# Autodesk Inventor assembly: wheel single_MIR
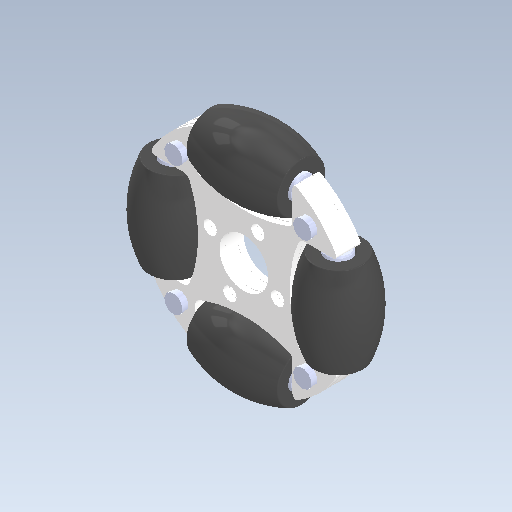
[picture p0: Inventor's stored thumbnail of the model, 512x512]
Saved by Autodesk Inventor 2020 (Build 240168000, 168)
## iProperties
Created: 2019-10-31
Part Number: wheel single_MIR
Document SubType Name: Assembly
Designer: jackm
Author: ball
Revision Number: ÈÎºÎ
## Documents named in this file (7)
- D:\FTC8863\2019 Robot\Odoemetry module\wheel single_MIR.iam
- D:\FTC8863\2019 Robot\Odoemetry module\1.5´ç90¶ÈÂÖ¹Ì¶¨°å_MIR1.ipt
- D:\FTC8863\2019 Robot\Odoemetry module\1.5´ç90¶ÈÂÖ¹Ì¶¨±ßÆ¬_MIR1.ipt
- D:\FTC8863\2019 Robot\Odoemetry module\1.5´ç90¶ÈÂÖÐ¡ÂÖÖá_MIR1.ipt
- D:\FTC8863\2019 Robot\Odoemetry module\1.5´ç90¶È»¡ÐÎÂÖ_MIR1.ipt
- D:\FTC8863\2019 Robot\Odoemetry module\1.5´ç90¶ÈÂÖÈü¸ÖÌ×_MIR1.ipt
- D:\FTC8863\2019 Robot\Odoemetry module\wheel rivet_MIR.ipt
## Components (23 placed, 6 different names)
1. 1.5´ç90¶ÈÂÖ¹Ì¶¨°å_MIR1:1 — Mate:1, Mate:3
2. 1.5´ç90¶ÈÂÖ¹Ì¶¨±ßÆ¬_MIR1:1 — Mate:2, Mate:8, Mate:6, Mate:5, Mate:4, Mate:7
3. 1.5´ç90¶ÈÂÖ¹Ì¶¨±ßÆ¬_MIR1:2
4. 1.5´ç90¶ÈÂÖÐ¡ÂÖÖá_MIR1:1
5. 1.5´ç90¶È»¡ÐÎÂÖ_MIR1:1
6. 1.5´ç90¶ÈÂÖÈü¸ÖÌ×_MIR1:1
7. 1.5´ç90¶ÈÂÖÈü¸ÖÌ×_MIR1:2
8. 1.5´ç90¶ÈÂÖÐ¡ÂÖÖá_MIR1:2
9. 1.5´ç90¶ÈÂÖÐ¡ÂÖÖá_MIR1:3
10. 1.5´ç90¶ÈÂÖÐ¡ÂÖÖá_MIR1:4
11. 1.5´ç90¶ÈÂÖÈü¸ÖÌ×_MIR1:3
12. 1.5´ç90¶ÈÂÖÈü¸ÖÌ×_MIR1:4
13. 1.5´ç90¶ÈÂÖÈü¸ÖÌ×_MIR1:5
14. 1.5´ç90¶ÈÂÖÈü¸ÖÌ×_MIR1:6
15. 1.5´ç90¶ÈÂÖÈü¸ÖÌ×_MIR1:7
16. 1.5´ç90¶ÈÂÖÈü¸ÖÌ×_MIR1:8
17. 1.5´ç90¶È»¡ÐÎÂÖ_MIR1:2
18. 1.5´ç90¶È»¡ÐÎÂÖ_MIR1:3
19. 1.5´ç90¶È»¡ÐÎÂÖ_MIR1:4
20. wheel rivet_MIR:1 — Mate:2, Mate:1
21. wheel rivet_MIR:2 — Mate:8, Mate:6
22. wheel rivet_MIR:3 — Mate:5, Mate:4
23. wheel rivet_MIR:4 — Mate:7, Mate:3
## Relationships (8: Mate 8)
- Mate:2: 1.5´ç90¶ÈÂÖ¹Ì¶¨±ßÆ¬_MIR1:1 ↔ wheel rivet_MIR:1
- Mate:1: 1.5´ç90¶ÈÂÖ¹Ì¶¨°å_MIR1:1 ↔ wheel rivet_MIR:1
- Mate:8: 1.5´ç90¶ÈÂÖ¹Ì¶¨±ßÆ¬_MIR1:1 ↔ wheel rivet_MIR:2
- Mate:6: 1.5´ç90¶ÈÂÖ¹Ì¶¨±ßÆ¬_MIR1:1 ↔ wheel rivet_MIR:2
- Mate:5: 1.5´ç90¶ÈÂÖ¹Ì¶¨±ßÆ¬_MIR1:1 ↔ wheel rivet_MIR:3
- Mate:4: 1.5´ç90¶ÈÂÖ¹Ì¶¨±ßÆ¬_MIR1:1 ↔ wheel rivet_MIR:3
- Mate:7: 1.5´ç90¶ÈÂÖ¹Ì¶¨±ßÆ¬_MIR1:1 ↔ wheel rivet_MIR:4
- Mate:3: 1.5´ç90¶ÈÂÖ¹Ì¶¨°å_MIR1:1 ↔ wheel rivet_MIR:4
